# Autodesk Inventor assembly: Assembly1
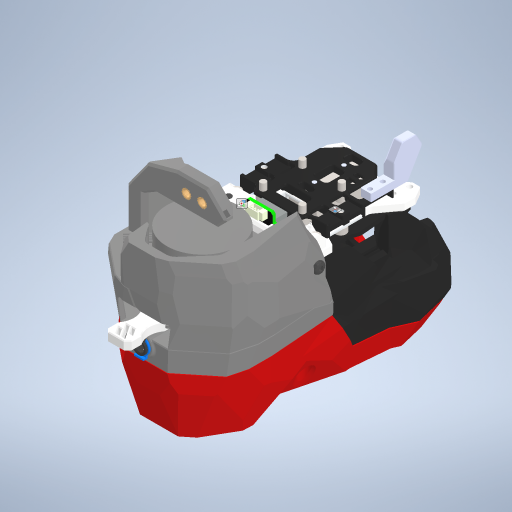
[picture p0: Inventor's stored thumbnail of the model, 512x512]
Saved by Autodesk Inventor 2024.2 (Build 282272000, 272)
## iProperties
Created: 2023-12-01
Part Number: Assembly1
Document SubType Name: Assembly
Designer: torban
Author: torban
## Documents named in this file (6)
- D:\GIT\Voron\Voron-Stealthburner\CAD\Cameron\Assembly1.iam
- D:\GIT\Voron\Voron-Stealthburner\CAD\Cameron\LGX_Lite_Stealthburner_ERCF_rev01\LGX_Lite_Stealthburner_ERCF_rev01.iam
- D:\GIT\Voron\Voron-Stealthburner\CAD\Cameron\Stealthburner_Printhead_Dragon.ipt
- D:\GIT\Voron\Voron-Stealthburner\CAD\Cameron\Stealthburner_CW2_Assembly\Stealthburner_CW2_Assembly.iam
- D:\GIT\Voron\Voron-Stealthburner\CAD\Cameron\CNC VORON TAP V1.0\CNC VORON TAP V1.0_TOP.iam
- D:\GIT\Voron\Voron-Stealthburner\CAD\Cameron\V2 Hall Sensor Adapter\V2 Hall Sensor Adapter.ipt
## Components (5 placed, 5 different names)
1. LGX_Lite_Stealthburner_ERCF_rev01:1 [sub-assembly] — Mate:1, Mate:2, Mate:3, Mate:4, Mate:5, Mate:6, Mate:8, Angle:1
2. Stealthburner_Printhead_Dragon:1 — Mate:1, Mate:2, Mate:3, Mate:7
3. Stealthburner_CW2_Assembly:1 [sub-assembly] — Mate:4, Mate:5, Mate:6
4. CNC VORON TAP V1.0_TOP:1 [sub-assembly] — Mate:7, Mate:8, Angle:1, Mate:9, Mate:10, Mate:11
5. V2 Hall Sensor Adapter:1 — Mate:9, Mate:10, Mate:11
## Relationships (12: Mate 11, Angle 1)
- Mate:1: LGX_Lite_Stealthburner_ERCF_rev01:1 ↔ Stealthburner_Printhead_Dragon:1
- Mate:2: LGX_Lite_Stealthburner_ERCF_rev01:1 ↔ Stealthburner_Printhead_Dragon:1
- Mate:3: LGX_Lite_Stealthburner_ERCF_rev01:1 ↔ Stealthburner_Printhead_Dragon:1
- Mate:4: LGX_Lite_Stealthburner_ERCF_rev01:1 ↔ Stealthburner_CW2_Assembly:1
- Mate:5: LGX_Lite_Stealthburner_ERCF_rev01:1 ↔ Stealthburner_CW2_Assembly:1
- Mate:6: LGX_Lite_Stealthburner_ERCF_rev01:1 ↔ Stealthburner_CW2_Assembly:1
- Mate:7: Stealthburner_Printhead_Dragon:1 ↔ CNC VORON TAP V1.0_TOP:1
- Mate:8: LGX_Lite_Stealthburner_ERCF_rev01:1 ↔ CNC VORON TAP V1.0_TOP:1
- Angle:1 (180 deg): LGX_Lite_Stealthburner_ERCF_rev01:1 ↔ CNC VORON TAP V1.0_TOP:1
- Mate:9: CNC VORON TAP V1.0_TOP:1 ↔ V2 Hall Sensor Adapter:1
- Mate:10: CNC VORON TAP V1.0_TOP:1 ↔ V2 Hall Sensor Adapter:1
- Mate:11: CNC VORON TAP V1.0_TOP:1 ↔ V2 Hall Sensor Adapter:1
